# Autodesk Inventor assembly: WheelieBar
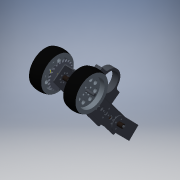
[picture p0: Inventor's stored thumbnail of the model, 180x180]
Saved by Autodesk Inventor 2016 (Build 200138000, 138)
## iProperties
Created: 2015-12-14
Part Number: WheelieBar
Document SubType Name: Assembly
Designer: tbloo
Author: tbloo
## Documents named in this file (12)
- C:\Users\tbloo\Documents\GitHub\phi_robotics\3d-models\FTC_Tetrix_KOP_Block_Party\Tim Bloot Designs\JAr JaR Bot\WheelieBar.iam
- C:\Users\tbloo\Documents\GitHub\phi_robotics\3d-models\FTC_Tetrix_KOP_Block_Party\Tetrix_Kit_FTC\Autodesk Inventor Files\tetrix_c_channel-3.ipt
- C:\Users\tbloo\Documents\GitHub\phi_robotics\3d-models\FTC_Tetrix_KOP_Block_Party\Tetrix_Kit_FTC\Autodesk Inventor Files\tetrix_axle.ipt
- C:\Users\tbloo\Documents\GitHub\phi_robotics\3d-models\FTC_Tetrix_KOP_Block_Party\Tetrix_Kit_FTC\Autodesk Inventor Files\tetrix_wheel-small.ipt
- C:\Users\tbloo\Documents\GitHub\phi_robotics\3d-models\FTC_Tetrix_KOP_Block_Party\Tetrix_Kit_FTC\Autodesk Inventor Files\tetrix_axle_lock.iam
- C:\Users\tbloo\Documents\GitHub\phi_robotics\3d-models\FTC_Tetrix_KOP_Block_Party\Tetrix_Kit_FTC\Autodesk Inventor Files\tetrix_chain_gear-24t.ipt
- C:\Users\tbloo\Documents\GitHub\phi_robotics\3d-models\FTC_Tetrix_KOP_Block_Party\Tetrix_Kit_FTC\Autodesk Inventor Files\tetrix_screw.ipt
- C:\Users\tbloo\Documents\GitHub\phi_robotics\3d-models\FTC_Tetrix_KOP_Block_Party\Tetrix_Kit_FTC\Autodesk Inventor Files\tetrix_bushing.ipt
- C:\Users\tbloo\Documents\GitHub\phi_robotics\3d-models\FTC_Tetrix_KOP_Block_Party\Tetrix_Kit_FTC\Autodesk Inventor Files\tetrix_axle_spacer-small.ipt
- C:\Users\tbloo\Documents\GitHub\phi_robotics\3d-models\FTC_Tetrix_KOP_Block_Party\Tetrix_Kit_FTC\Autodesk Inventor Files\tetrix_motor_mount-old.ipt
- C:\Users\tbloo\Documents\GitHub\phi_robotics\3d-models\FTC_Tetrix_KOP_Block_Party\Tetrix_Kit_FTC\Autodesk Inventor Files\tetrix_739063_2012.ipt
- C:\Users\tbloo\Documents\GitHub\phi_robotics\3d-models\FTC_Tetrix_KOP_Block_Party\Tetrix_Kit_FTC\Autodesk Inventor Files\tetrix_axle_spacer_mount.ipt
## Components (21 placed, 11 different names)
1. tetrix_c_channel-3:1 — Rotational:1, Rotational:2, Rigid:8, Rotational:9, Rotational:10
2. tetrix_axle:1 — Rigid:5
3. tetrix_wheel-small:1 — Rigid:7
4. tetrix_wheel-small:2 — Rigid:1, Rotational:3
5. tetrix_axle_lock:2 [sub-assembly] — Rigid:2, Rigid:6
6. tetrix_chain_gear-24t:1 — Rigid:2, Rigid:3, Rigid:4, Rotational:4
7. tetrix_axle_lock:3 [sub-assembly] — Rigid:1, Rigid:5
8. tetrix_screw:1 — Rigid:3
9. tetrix_screw:2 — Rigid:4
10. tetrix_bushing:1 — Rotational:1, Rotational:5
11. tetrix_bushing:2 — Rotational:2, Rotational:6
12. tetrix_axle_spacer-small:1 — Rotational:3, Rigid:6
13. tetrix_axle_spacer-small:2 — Rotational:4, Rotational:5
14. tetrix_axle_lock:4 [sub-assembly] — Rigid:7, Rotational:7
15. tetrix_axle_spacer-small:3 — Rotational:6, Rotational:7
16. tetrix_motor_mount-old:1 — Rigid:8
17. tetrix_739063_2012:1 — Rotational:8, Rotational:11
18. tetrix_axle_spacer_mount:1 — Rotational:8, Rotational:9, Rotational:12
19. tetrix_axle:2 — Rotational:12
20. tetrix_bushing:3 — Rotational:11
21. tetrix_bushing:4 — Rotational:10
## Relationships (20: RevoluteJoint 12, WeldJoint 8)
- Rigid:1 [WeldJoint]: tetrix_wheel-small:2 ↔ tetrix_axle_lock:3
- Rigid:2 [WeldJoint]: tetrix_axle_lock:2 ↔ tetrix_chain_gear-24t:1
- Rigid:3 [WeldJoint]: tetrix_chain_gear-24t:1 ↔ tetrix_screw:1
- Rigid:4 [WeldJoint]: tetrix_chain_gear-24t:1 ↔ tetrix_screw:2
- Rotational:1 [RevoluteJoint]: tetrix_c_channel-3:1 ↔ tetrix_bushing:1
- Rotational:2 [RevoluteJoint]: tetrix_c_channel-3:1 ↔ tetrix_bushing:2
- Rigid:5 [WeldJoint]: tetrix_axle:1 ↔ tetrix_axle_lock:3
- Rotational:3 [RevoluteJoint]: tetrix_wheel-small:2 ↔ tetrix_axle_spacer-small:1
- Rigid:6 [WeldJoint]: tetrix_axle_lock:2 ↔ tetrix_axle_spacer-small:1
- Rotational:4 [RevoluteJoint]: tetrix_chain_gear-24t:1 ↔ tetrix_axle_spacer-small:2
- Rotational:5 [RevoluteJoint]: tetrix_bushing:1 ↔ tetrix_axle_spacer-small:2
- Rigid:7 [WeldJoint]: tetrix_wheel-small:1 ↔ tetrix_axle_lock:4
- Rotational:6 [RevoluteJoint]: tetrix_bushing:2 ↔ tetrix_axle_spacer-small:3
- Rotational:7 [RevoluteJoint]: tetrix_axle_lock:4 ↔ tetrix_axle_spacer-small:3
- Rigid:8 [WeldJoint]: tetrix_c_channel-3:1 ↔ tetrix_motor_mount-old:1
- Rotational:8 [RevoluteJoint]: tetrix_739063_2012:1 ↔ tetrix_axle_spacer_mount:1
- Rotational:9 [RevoluteJoint]: tetrix_c_channel-3:1 ↔ tetrix_axle_spacer_mount:1
- Rotational:10 [RevoluteJoint]: tetrix_c_channel-3:1 ↔ tetrix_bushing:4
- Rotational:11 [RevoluteJoint]: tetrix_739063_2012:1 ↔ tetrix_bushing:3
- Rotational:12 [RevoluteJoint]: tetrix_axle_spacer_mount:1 ↔ tetrix_axle:2
